# Autodesk Inventor assembly: 22925T72
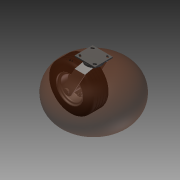
[picture p0: Inventor's stored thumbnail of the model, 180x180]
Saved by Autodesk Inventor 2016 (Build 200138000, 138)
## iProperties
Created: 2016-04-01
Part Number: 22925T72
Document SubType Name: Assembly
Designer: hwasserb
Author: hwasserb
## Documents named in this file (4)
- C:\Users\Haden\Desktop\Cad-Model\Rear Wheel\22925T72.iam
- C:\Users\Haden\Desktop\Cad-Model\Rear Wheel\Pneumatic Tire.ipt
- C:\Users\Haden\Desktop\Cad-Model\Rear Wheel\Caster.ipt
- C:\Users\Haden\Desktop\Cad-Model\Rear Wheel\Rear Wheel Radius.ipt
## Components (3 placed, 3 different names)
1. Pneumatic Tire:1 — Mate:1, Mate:2
2. Caster:1 — Mate:1, Mate:2, Mate:3, Mate:4
3. Rear Wheel Radius:1 — Mate:3, Mate:4
## Relationships (4: Mate 4)
- Mate:1: Pneumatic Tire:1 ↔ Caster:1
- Mate:2 (2.54 mm): Pneumatic Tire:1 ↔ Caster:1
- Mate:3 (44.45 mm): Caster:1 ↔ Rear Wheel Radius:1
- Mate:4: Caster:1 ↔ Rear Wheel Radius:1
